# Autodesk Inventor assembly: PD Rev 3 PCB
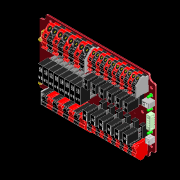
[picture p0: Inventor's stored thumbnail of the model, 180x180]
Saved by Autodesk Inventor 2012 (Build 160160000, 160)
## iProperties
Company: Team 801
Created: 2008-05-31
Part Number: PD Rev 3 PCB
Document SubType Name: Assembly
Designer: Jeffrey M
Catalog Web Link: www.team801.org
Mass: 388.452 g
Surface Area: 2329.68 cm^2
Volume: 368.95 cm^3
Density: 1.05286 g/cm^3
Translation Standard: STEP AP214IS
File Name: Open CASCADE Shape Model
Preprocessor: Open CASCADE 6.2
Postprocessor: Build: 320, Release: 2008 SP2 - Date: Mon 11/26/2007
Sent Units: MILLIMETERS
Uncertainty: 2e-06
Author: Jeffrey M
## Documents named in this file (11)
- Z:\UserData\Documents\Inventor\team1885frc\Electronics\PowerDistributionBoard\PD Rev3 PCB.iam
- Z:\UserData\Documents\Inventor\team1885frc\Electronics\PowerDistributionBoard\PD Rev3 Board.ipt
- Z:\UserData\Documents\Inventor\team1885frc\Electronics\PowerDistributionBoard\Wago 745-831 (32A) Block.iam
- Z:\UserData\Documents\Inventor\team1885frc\Electronics\PowerDistributionBoard\Wago 745-851 (76A) Block.iam
- Z:\UserData\Documents\Inventor\team1885frc\Electronics\PowerDistributionBoard\LED.ipt
- Z:\UserData\Documents\Inventor\team1885frc\Electronics\PowerDistributionBoard\Big CB in Holder.ipt
- Z:\UserData\Documents\Inventor\team1885frc\Electronics\PowerDistributionBoard\Medium CB in Holder.ipt
- Z:\UserData\Documents\Inventor\team1885frc\Electronics\PowerDistributionBoard\Wurth Lug.ipt
- Z:\UserData\Documents\Inventor\team1885frc\Electronics\PowerDistributionBoard\Wago 734-132.ipt
- Z:\UserData\Documents\Inventor\team1885frc\Electronics\PowerDistributionBoard\Wago 739-302.ipt
- Z:\UserData\Documents\Inventor\team1885frc\Electronics\PowerDistributionBoard\CTM040V8.ipt
## Components (33 placed, 10 different names)
1. PD Rev3 Board:1 — Mate:1, Mate:2, Mate:3, Mate:4, Mate:5, Mate:6, Mate:7, Mate:8, Mate:9, Mate:10, Mate:13, Mate:16, Mate:19, Mate:22, Mate:24, Mate:26, Mate:27, Mate:28, Mate:29, Mate:32, Mate:35, Mate:36, Mate:37, Mate:38, Mate:39, Mate:40, Mate:41, Mate:42, Mate:43, Mate:44, Mate:45, Mate:46, Mate:47, Mate:48, Mate:49, Mate:50, Mate:51
2. Wago 745-831 (32A) Block:1 [sub-assembly] — Mate:1, Mate:2, Mate:3
3. Wago 745-831 (32A) Block:2 [sub-assembly] — Mate:4, Mate:5, Mate:6
4. Wago 745-851 (76A) Block:1 [sub-assembly] — Mate:10, Mate:37, Mate:38
5. Wago 745-851 (76A) Block:2 [sub-assembly] — Mate:7, Mate:8, Mate:9
6. LED:1 — Mate:13, Mate:48, Mate:49
7. LED:2 — Mate:16, Mate:41, Mate:42
8. 734-132:1 — Mate:29, Mate:46, Mate:47
9. LED:3 — Mate:19, Mate:39, Mate:40
10. Wurth Lug:1 — Mate:22, Angle:1, Mate:50
11. Wurth Lug:2 — Mate:24, Angle:2, Mate:51
12. 739-302:1 — Mate:32, Mate:43, Mate:44
13. CTM040V8:1 — Mate:35, Mate:36, Mate:45
14. Big CB in Holder:1 — Mate:26
15. Big CB in Holder:2
16. Big CB in Holder:3
17. Big CB in Holder:4
18. Big CB in Holder:5
19. Big CB in Holder:6
20. Big CB in Holder:7
21. Big CB in Holder:8
22. Medium CB in Holder:2 — Mate:28
23. Medium CB in Holder:1 — Mate:27
24. Medium CB in Holder:3
25. Medium CB in Holder:4
26. Medium CB in Holder:5
27. Medium CB in Holder:6
28. Medium CB in Holder:7
29. Medium CB in Holder:8
30. Medium CB in Holder:9
31. Medium CB in Holder:10
32. Medium CB in Holder:11
33. Medium CB in Holder:12
## Component patterns: (8 elements, first: Big CB in Holder:1), (6 elements, first: Medium CB in Holder:2 + Medium CB in Holder:1)
## Relationships (39: Mate 37, Angle 2)
- Mate:1: PD Rev3 Board:1 ↔ Wago 745-831 (32A) Block:1
- Mate:2: PD Rev3 Board:1 ↔ Wago 745-831 (32A) Block:1
- Mate:3: PD Rev3 Board:1 ↔ Wago 745-831 (32A) Block:1
- Mate:4: PD Rev3 Board:1 ↔ Wago 745-831 (32A) Block:2
- Mate:5: PD Rev3 Board:1 ↔ Wago 745-831 (32A) Block:2
- Mate:6: PD Rev3 Board:1 ↔ Wago 745-831 (32A) Block:2
- Mate:7: PD Rev3 Board:1 ↔ Wago 745-851 (76A) Block:2
- Mate:8: PD Rev3 Board:1 ↔ Wago 745-851 (76A) Block:2
- Mate:9: PD Rev3 Board:1 ↔ Wago 745-851 (76A) Block:2
- Mate:10: PD Rev3 Board:1 ↔ Wago 745-851 (76A) Block:1
- Mate:13: PD Rev3 Board:1 ↔ LED:1
- Mate:16: PD Rev3 Board:1 ↔ LED:2
- Mate:19: PD Rev3 Board:1 ↔ LED:3
- Mate:22: PD Rev3 Board:1 ↔ Wurth Lug:1
- Angle:1 (180 deg): Wurth Lug:1
- Mate:24: PD Rev3 Board:1 ↔ Wurth Lug:2
- Angle:2 (180 deg): Wurth Lug:2
- Mate:26 (3.2766 mm): PD Rev3 Board:1 ↔ Big CB in Holder:1
- Mate:27: PD Rev3 Board:1 ↔ Medium CB in Holder:1
- Mate:28: PD Rev3 Board:1 ↔ Medium CB in Holder:2
- Mate:29: PD Rev3 Board:1 ↔ 734-132:1
- Mate:32: PD Rev3 Board:1 ↔ 739-302:1
- Mate:35: PD Rev3 Board:1 ↔ CTM040V8:1
- Mate:36: PD Rev3 Board:1 ↔ CTM040V8:1
- Mate:37: PD Rev3 Board:1 ↔ Wago 745-851 (76A) Block:1
- Mate:38: PD Rev3 Board:1 ↔ Wago 745-851 (76A) Block:1
- Mate:39: PD Rev3 Board:1 ↔ LED:3
- Mate:40: PD Rev3 Board:1 ↔ LED:3
- Mate:41: PD Rev3 Board:1 ↔ LED:2
- Mate:42: PD Rev3 Board:1 ↔ LED:2
- Mate:43: PD Rev3 Board:1 ↔ 739-302:1
- Mate:44: PD Rev3 Board:1 ↔ 739-302:1
- Mate:45: PD Rev3 Board:1 ↔ CTM040V8:1
- Mate:46: PD Rev3 Board:1 ↔ 734-132:1
- Mate:47: PD Rev3 Board:1 ↔ 734-132:1
- Mate:48: PD Rev3 Board:1 ↔ LED:1
- Mate:49: PD Rev3 Board:1 ↔ LED:1
- Mate:50: PD Rev3 Board:1 ↔ Wurth Lug:1
- Mate:51: PD Rev3 Board:1 ↔ Wurth Lug:2
